# Autodesk Inventor assembly: MaleHeaderPin_1x2_90
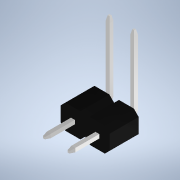
[picture p0: Inventor's stored thumbnail of the model, 180x180]
Saved by Autodesk Inventor 2021 (Build 250183000, 183)
## iProperties
Created: 2021-07-24
Part Number: MaleHeaderPin_1x2_90
Document SubType Name: Assembly
Designer: ermoz
Author: ermoz
## Documents named in this file (2)
- D:\Moje Wyczyny\My_Poor_Projects\Sneak100_MiniSumo\minisumo-sneak100\mechanics\ElectricElements\MaleHeaderPin_1x2_90.iam
- D:\Moje Wyczyny\My_Poor_Projects\Sneak100_MiniSumo\minisumo-sneak100\mechanics\ElectricElements\MaleHeaderPin_90.ipt
## Components (2 placed, 1 different names)
1. MaleHeaderPin_90:1 — Mate:1, Flush:1, Flush:6
2. MaleHeaderPin_90:2 — Mate:1, Flush:1, Flush:6
## Relationships (3: Flush 2, Mate 1)
- Mate:1: MaleHeaderPin_90:1 ↔ MaleHeaderPin_90:2
- Flush:1: MaleHeaderPin_90:1 ↔ MaleHeaderPin_90:2
- Flush:6: MaleHeaderPin_90:1 ↔ MaleHeaderPin_90:2
